# Autodesk Inventor assembly: sunon_fan_red
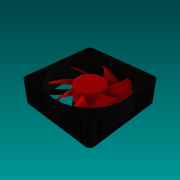
[picture p0: Inventor's stored thumbnail of the model, 180x180]
Saved by Autodesk Inventor 2015 (Build 190159000, 159)
## iProperties
Created: 2015-03-08
Part Number: sunon_fan_red
Document SubType Name: Assembly
Designer: Venci
Author: Venci
## Documents named in this file (3)
- C:\Users\Venci\Google Drive\Inventor Projects\FAN\80mm\sunon_fan_red.iam
- C:\Users\Venci\Google Drive\Inventor Projects\FAN\80mm\sunon_frame.ipt
- C:\Users\Venci\Google Drive\Inventor Projects\FAN\80mm\sunon_blade_80.ipt
## Components (2 placed, 2 different names)
1. sunon_frame:1 — Insert:1
2. sunon_blade_80:1 — Insert:1
## Relationships (1: Insert 1)
- Insert:1: sunon_frame:1 ↔ sunon_blade_80:1
